# Autodesk Inventor assembly: Eslabon1
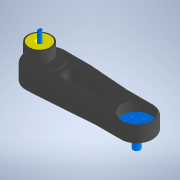
[picture p0: Inventor's stored thumbnail of the model, 180x180]
Saved by Autodesk Inventor 2021 (Build 250183000, 183)
## iProperties
Created: 2022-04-22
Part Number: Eslabon1
Document SubType Name: Assembly
Designer: Alcatraz
Author: Alcatraz
## Documents named in this file (7)
- F:\Tesis\TESIS\Matlab\Pruebas\Prueba3_Simulacion1\Eslabon1.iam
- F:\Tesis\TESIS\Eslabon_9_Parametrizado.ipt
- F:\Tesis\TESIS\Tapa_eslabon.ipt
- F:\Tesis\TESIS\AX-12A,18A,12W,MX-12W(stp)\AX-12A.iam
- F:\Tesis\TESIS\rodamiento_dummie.ipt
- F:\Tesis\TESIS\Brida_5_parametrizado.ipt
- F:\Tesis\TESIS\Eje_3_parametrizado.ipt
## Components (7 placed, 6 different names)
1. Eslabon_9_Parametrizado:1 — Coincidencia:1, Coincidencia:5, Coincidencia:6, Coincidencia:7, Coincidencia:13, Coincidencia:14, Coincidencia:15, Coincidencia:16, Coincidencia:17
2. Tapa_eslabon:1 — Coincidencia:1, Coincidencia:2, Coincidencia:3, Coincidencia:4, Coincidencia:5, Coincidencia:6, Coincidencia:7
3. AX-12A:1 [sub-assembly] — Coincidencia:2, Coincidencia:3, Coincidencia:4, Coincidencia:10, Coincidencia:11, Coincidencia:12
4. rodamiento_dummie:1 — Coincidencia:8, Coincidencia:9, Coincidencia:14
5. rodamiento_dummie:2 — Coincidencia:8, Coincidencia:9, Coincidencia:13
6. Brida_5_parametrizado:1 — Coincidencia:10, Coincidencia:11, Coincidencia:12
7. Eje_3_parametrizado:1 — Coincidencia:15, Coincidencia:16, Coincidencia:17
## Relationships (17: Mate 17)
- Coincidencia:1 [Mate]: Eslabon_9_Parametrizado:1 ↔ Tapa_eslabon:1
- Coincidencia:2 [Mate]: Tapa_eslabon:1 ↔ AX-12A:1
- Coincidencia:3 [Mate]: Tapa_eslabon:1 ↔ AX-12A:1
- Coincidencia:4 [Mate]: Tapa_eslabon:1 ↔ AX-12A:1
- Coincidencia:5 [Mate]: Eslabon_9_Parametrizado:1 ↔ Tapa_eslabon:1
- Coincidencia:6 [Mate]: Eslabon_9_Parametrizado:1 ↔ Tapa_eslabon:1
- Coincidencia:7 [Mate]: Eslabon_9_Parametrizado:1 ↔ Tapa_eslabon:1
- Coincidencia:8 [Mate]: rodamiento_dummie:1 ↔ rodamiento_dummie:2
- Coincidencia:9 [Mate]: rodamiento_dummie:1 ↔ rodamiento_dummie:2
- Coincidencia:10 [Mate]: AX-12A:1 ↔ Brida_5_parametrizado:1
- Coincidencia:11 [Mate]: AX-12A:1 ↔ Brida_5_parametrizado:1
- Coincidencia:12 [Mate]: AX-12A:1 ↔ Brida_5_parametrizado:1
- Coincidencia:13 [Mate]: Eslabon_9_Parametrizado:1 ↔ rodamiento_dummie:2
- Coincidencia:14 [Mate]: Eslabon_9_Parametrizado:1 ↔ rodamiento_dummie:1
- Coincidencia:15 [Mate]: Eslabon_9_Parametrizado:1 ↔ Eje_3_parametrizado:1
- Coincidencia:16 [Mate]: Eslabon_9_Parametrizado:1 ↔ Eje_3_parametrizado:1
- Coincidencia:17 [Mate]: Eslabon_9_Parametrizado:1 ↔ Eje_3_parametrizado:1
